# Autodesk Inventor assembly: Vini-MyPnP
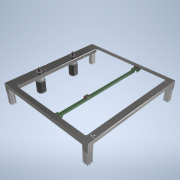
[picture p0: Inventor's stored thumbnail of the model, 180x180]
Saved by Autodesk Inventor 2020 (Build 240168000, 168)
## iProperties
Created: 2020-03-06
Part Number: Vini-MyPnP
Document SubType Name: Assembly
Designer: 10300812
Author: 10300812
## Documents named in this file (7)
- C:\Users\10300812\Documents\GitHub\MyPnP\Vini-MyPnP.iam
- C:\Users\10300812\Documents\GitHub\MyPnP\Gantry.ipt
- C:\Users\10300812\Documents\GitHub\MyPnP\User Library-8-AS-6-4040-VSLOT.ipt
- C:\Users\10300812\Documents\GitHub\MyPnP\Y-Axis-Frame.ipt
- C:\Users\10300812\Documents\GitHub\MyPnP\Hiwin\MGN12C1R0053Z0CM-No-Set-E1_10_0_2_03.iam
- C:\Users\10300812\Documents\GitHub\MyPnP\bg-65sx25-885660110101.ipt
- C:\Users\10300812\Documents\GitHub\MyPnP\plg-63-8886301102.ipt
## Components (13 placed, 6 different names)
1. Gantry:1 — Mate:1, Mate:2, Mate:3, Mate:4, Mate:5, Mate:6, Mate:7, Mate:8, Flush:4, Mate:9, Mate:10, Mate:11, Mate:18, Mate:21, Mate:22, Mate:25, Mate:26, Mate:27, Mate:28, Angle:1, Angle:2
2. User Library-8-AS-6-4040-VSLOT:1 — Mate:1, Mate:2, Flush:2, Flush:3, Flush:4
3. User Library-8-AS-6-4040-VSLOT:2 — Mate:3, Mate:4, Flush:3
4. User Library-8-AS-6-4040-VSLOT:3 — Mate:5, Mate:6, Flush:1
5. User Library-8-AS-6-4040-VSLOT:4 — Mate:7, Mate:8, Flush:1, Flush:2
6. Y-Axis-Frame:1 — Mate:12, Mate:13, Mate:14, Mate:15, Mate:16, Mate:17, Mate:29, Mate:30, Mate:31
7. MGN12C1R0053Z0CM-No-Set-E1_10_0_2_03:1 [sub-assembly] — Mate:9, Mate:10, Mate:11, Mate:12, Mate:13, Mate:14
8. MGN12C1R0053Z0CM-No-Set-E1_10_0_2_03:2 [sub-assembly] — Mate:15, Mate:16, Mate:17, Mate:18
9. bg-65sx25-885660110101:1 — Mate:19, Mate:20, Angle:2
10. plg-63-8886301102:1 — Mate:19, Mate:20, Mate:21, Mate:22, Mate:28
11. bg-65sx25-885660110101:2 — Angle:1
12. plg-63-8886301102:2 — Mate:25, Mate:26, Mate:27
13. MGN12C1R0053Z0CM-No-Set-E1_10_0_2_03:3 [sub-assembly] — Mate:29, Mate:30, Mate:31
## Relationships (37: Mate 31, Flush 4, Angle 2)
- Mate:1: Gantry:1 ↔ User Library-8-AS-6-4040-VSLOT:1
- Mate:2: Gantry:1 ↔ User Library-8-AS-6-4040-VSLOT:1
- Mate:3: Gantry:1 ↔ User Library-8-AS-6-4040-VSLOT:2
- Mate:4: Gantry:1 ↔ User Library-8-AS-6-4040-VSLOT:2
- Mate:5: Gantry:1 ↔ User Library-8-AS-6-4040-VSLOT:3
- Mate:6: Gantry:1 ↔ User Library-8-AS-6-4040-VSLOT:3
- Mate:7: Gantry:1 ↔ User Library-8-AS-6-4040-VSLOT:4
- Mate:8: Gantry:1 ↔ User Library-8-AS-6-4040-VSLOT:4
- Flush:1: User Library-8-AS-6-4040-VSLOT:3 ↔ User Library-8-AS-6-4040-VSLOT:4
- Flush:2: User Library-8-AS-6-4040-VSLOT:1 ↔ User Library-8-AS-6-4040-VSLOT:4
- Flush:3: User Library-8-AS-6-4040-VSLOT:1 ↔ User Library-8-AS-6-4040-VSLOT:2
- Flush:4 (-100 mm): Gantry:1 ↔ User Library-8-AS-6-4040-VSLOT:1
- Mate:9: Gantry:1 ↔ MGN12C1R0053Z0CM-No-Set-E1_10_0_2_03:1
- Mate:10: Gantry:1 ↔ MGN12C1R0053Z0CM-No-Set-E1_10_0_2_03:1
- Mate:11: Gantry:1 ↔ MGN12C1R0053Z0CM-No-Set-E1_10_0_2_03:1
- Mate:12: Y-Axis-Frame:1 ↔ MGN12C1R0053Z0CM-No-Set-E1_10_0_2_03:1
- Mate:13: Y-Axis-Frame:1 ↔ MGN12C1R0053Z0CM-No-Set-E1_10_0_2_03:1
- Mate:14: Y-Axis-Frame:1 ↔ MGN12C1R0053Z0CM-No-Set-E1_10_0_2_03:1
- Mate:15: Y-Axis-Frame:1 ↔ MGN12C1R0053Z0CM-No-Set-E1_10_0_2_03:2
- Mate:16: Y-Axis-Frame:1 ↔ MGN12C1R0053Z0CM-No-Set-E1_10_0_2_03:2
- Mate:17: Y-Axis-Frame:1 ↔ MGN12C1R0053Z0CM-No-Set-E1_10_0_2_03:2
- Mate:18: Gantry:1 ↔ MGN12C1R0053Z0CM-No-Set-E1_10_0_2_03:2
- Mate:19: bg-65sx25-885660110101:1 ↔ plg-63-8886301102:1
- Mate:20: bg-65sx25-885660110101:1 ↔ plg-63-8886301102:1
- Mate:21: Gantry:1 ↔ plg-63-8886301102:1
- Mate:22: Gantry:1 ↔ plg-63-8886301102:1
- [Mate]: bg-65sx25-885660110101:2 ↔ plg-63-8886301102:2
- [Mate]: bg-65sx25-885660110101:2 ↔ plg-63-8886301102:2
- Mate:25: Gantry:1 ↔ plg-63-8886301102:2
- Mate:26: Gantry:1 ↔ plg-63-8886301102:2
- Mate:27: Gantry:1 ↔ plg-63-8886301102:2
- Mate:28: Gantry:1 ↔ plg-63-8886301102:1
- Angle:1 (0 deg): Gantry:1 ↔ bg-65sx25-885660110101:2
- Angle:2 (0 deg): Gantry:1 ↔ bg-65sx25-885660110101:1
- Mate:29: Y-Axis-Frame:1 ↔ MGN12C1R0053Z0CM-No-Set-E1_10_0_2_03:3
- Mate:30: Y-Axis-Frame:1 ↔ MGN12C1R0053Z0CM-No-Set-E1_10_0_2_03:3
- Mate:31: Y-Axis-Frame:1 ↔ MGN12C1R0053Z0CM-No-Set-E1_10_0_2_03:3
## Named parameters: d26_d22 = 0 mm, d27_d23 = 0 mm
